# Autodesk Inventor assembly: attachmentCircularEnsamble
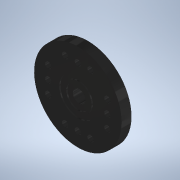
[picture p0: Inventor's stored thumbnail of the model, 180x180]
Saved by Autodesk Inventor 2020.3 (Build 243373000, 373)
## iProperties
Created: 2020-11-02
Part Number: attachmentCircularEnsamble
Document SubType Name: Assembly
Designer: juanp
Author: juanp
## Documents named in this file (3)
- C:\Users\juanp\Desktop\Diseño EVA\Dispensador\Servo MG996R\attachmentCircularEnsamble.iam
- C:\Users\juanp\Desktop\Diseño EVA\Dispensador\Servo MG996R\attachmentCircular.ipt
- C:\Users\juanp\Desktop\Diseño EVA\Dispensador\Servo MG996R\attachmentCircular_1.ipt
## Components (2 placed, 2 different names)
1. attachmentCircular:1 — Mate:1, Mate:2
2. attachmentCircular_1:1 — Mate:1, Mate:2
## Relationships (2: Mate 2)
- Mate:1: attachmentCircular:1 ↔ attachmentCircular_1:1
- Mate:2: attachmentCircular:1 ↔ attachmentCircular_1:1
